# Autodesk Inventor assembly: complete
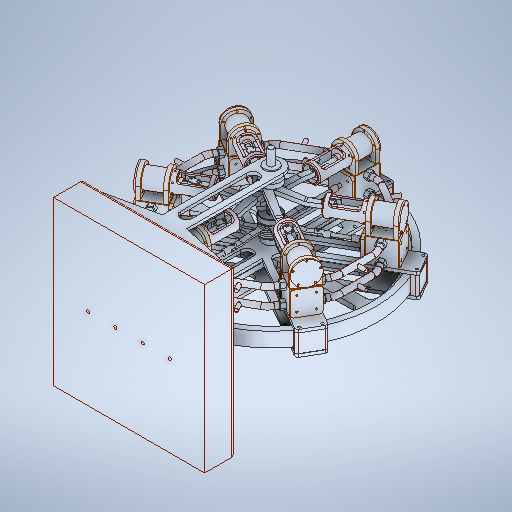
[picture p0: Inventor's stored thumbnail of the model, 512x512]
Saved by Autodesk Inventor 2025.1 (Build 291241000, 241)
## iProperties
Created: 2024-09-18
Part Number: complete
Document SubType Name: Assembly
Designer: ffogue
Author: ffogue
## Documents named in this file (23)
- C:\Users\ffogue\Documents\Inventor\Cylinder Radial Steam Engine\complete.iam
- C:\Users\ffogue\Documents\Inventor\Cylinder Radial Steam Engine\03.ipt
- C:\Users\ffogue\Documents\Inventor\Cylinder Radial Steam Engine\02A.ipt
- C:\Users\ffogue\Documents\Inventor\Cylinder Radial Steam Engine\05.ipt
- C:\Users\ffogue\Documents\Inventor\Cylinder Radial Steam Engine\04.ipt
- C:\Users\ffogue\Documents\Inventor\Cylinder Radial Steam Engine\08.ipt
- C:\Users\ffogue\Documents\Inventor\Cylinder Radial Steam Engine\09.ipt
- C:\Users\ffogue\Documents\Inventor\Cylinder Radial Steam Engine\Block.ipt
- C:\Users\ffogue\Documents\Inventor\Cylinder Radial Steam Engine\02.ipt
- C:\Users\ffogue\Documents\Inventor\Cylinder Radial Steam Engine\03A.ipt
- C:\Users\ffogue\Documents\Inventor\Cylinder Radial Steam Engine\block.iam
- C:\Users\ffogue\Documents\Inventor\Cylinder Radial Steam Engine\51.ipt
- C:\Users\ffogue\Documents\Inventor\Cylinder Radial Steam Engine\axis.iam
- C:\Users\ffogue\Documents\Inventor\Cylinder Radial Steam Engine\axis assembly.iam
- C:\Users\ffogue\Documents\Inventor\Cylinder Radial Steam Engine\15_3.iam
- C:\Users\ffogue\Documents\Inventor\Cylinder Radial Steam Engine\15_2.iam
- C:\Users\ffogue\Documents\Inventor\Cylinder Radial Steam Engine\15_1.iam
- C:\Users\ffogue\Documents\Inventor\Cylinder Radial Steam Engine\11.ipt
- C:\Users\ffogue\Documents\Inventor\Cylinder Radial Steam Engine\12.ipt
- C:\Users\ffogue\Documents\Inventor\Cylinder Radial Steam Engine\47.ipt
- C:\Users\ffogue\Documents\Inventor\Cylinder Radial Steam Engine\47B.ipt
- C:\Users\ffogue\Documents\Inventor\Cylinder Radial Steam Engine\47A.ipt
- C:\Users\ffogue\Documents\Inventor\Cylinder Radial Steam Engine\Welle.iam
## Components (68 placed, 22 different names)
1. 03:1 — Mate:1, Mate:3, Insert:2, Mate:14, Mate:18, Insert:12, Insert:13, Insert:14, Mate:27, Insert:21, Mate:109, Insert:38
2. 03:2 — Mate:1, Flush:1, Flush:2, Mate:2, Insert:1, Mate:4, Mate:15, Mate:16, Mate:17, Mate:22, Mate:23, Insert:11, Mate:24, Mate:25, Mate:26, Insert:15, Insert:20, Mate:110, Insert:39
3. 02A:1 — Flush:1, Flush:2, Mate:2, Insert:1, Mate:3, Insert:2
4. 05:1 — Mate:4, Mate:5, Mate:6, Insert:5, Insert:6, Mate:7, Mate:8, Angle:1, Rotation:1, Rotation:2
5. 08:1 — Mate:6, Insert:5, Mate:8, Mate:9, Mate:10, Mate:11, Mate:12, Flush:3, Flush:4, Flush:5, Flush:6, Insert:22
6. 08:2 — Mate:5, Insert:6, Mate:7
7. 09:1 — Mate:9, Flush:6
8. 09:2 — Mate:10, Flush:4
9. 09:3 — Mate:12, Flush:3
10. 09:4 — Mate:11, Flush:5
11. Block:1 — Mate:13, Insert:7, Angle:2
12. 02:1 — Mate:13, Insert:7, Mate:14, Mate:15, Mate:16, Mate:17, Mate:18, Mate:19, Insert:8
13. 03A:1 — Mate:19, Insert:8, Insert:10, Mate:148, Insert:54
14. 04:3 — Insert:10
15. 02A:2 — Mate:24, Insert:12
16. 02A:3 — Mate:25, Insert:13
17. 02A:4 — Mate:27, Insert:15
18. 02A:5 — Mate:26, Insert:14
19. 04:5 — Insert:21
20. 04:6 — Insert:20, Insert:22
21. axis:1 [sub-assembly] — Mate:61, Mate:130, Insert:45
22. axis assembly:1 [sub-assembly] — Mate:66, Mate:104, Insert:35
23. axis assembly:2 [sub-assembly] — Mate:75, Mate:99, Insert:33
24. axis assembly:3 [sub-assembly] — Mate:77, Mate:108, Insert:37
25. axis assembly:4 [sub-assembly] — Mate:80, Mate:97, Insert:32
26. axis assembly:5 [sub-assembly] — Mate:89, Mate:95, Insert:31
27. 15_3:2 [sub-assembly] — Mate:95, Insert:31, Mate:96, Mate:105, Mate:107
28. 15_3:3 [sub-assembly] — Mate:96, Mate:97, Insert:32, Mate:98, Mate:103, Mate:113, Insert:42
29. 15_2:1 [sub-assembly] — Mate:98, Mate:99, Insert:33
30. axis assembly:6 [sub-assembly] — Mate:101, Mate:106, Insert:36
31. 15_1:2 [sub-assembly] — Mate:103, Mate:104, Insert:35
32. 15_1:3 [sub-assembly] — Mate:105, Mate:106, Insert:36
33. 15_2:2 [sub-assembly] — Mate:107, Mate:108, Insert:37
34. 08:3 — Mate:109, Insert:38
35. 08:4 — Mate:110, Insert:39, Mate:114, Mate:150
36. 11:1 — Mate:111, Mate:112, Insert:40, Insert:41, Mate:113, Mate:114
37. 12:1 — Mate:112, Insert:41, Insert:42, Mate:116, Mate:149
38. 12:2 — Mate:111, Insert:40, Mate:116, Rotation:2
39. axis:2 [sub-assembly] — Mate:117, Mate:133, Insert:51
40. axis:3 [sub-assembly] — Mate:118, Mate:143, Insert:52
41. axis:4 [sub-assembly] — Mate:119, Mate:129, Insert:44
42. axis:5 [sub-assembly] — Mate:120, Mate:141, Insert:50
43. axis:6 [sub-assembly] — Mate:121, Mate:145, Insert:53
44. 47:1 — Mate:123, Mate:129, Insert:44
45. 47:2 — Mate:123, Mate:130, Insert:45, Mate:140
46. 47B:1 — Mate:133, Insert:51, Mate:142
47. 47B:2 — Mate:140, Mate:141, Insert:50, Mate:144
48. 47A:1 — Mate:142, Mate:143, Insert:52, Mate:146, Mate:147
49. 47A:2 — Mate:144, Mate:145, Insert:53, Mate:146
50. Welle:1 [sub-assembly] — Mate:147, Mate:148, Mate:149, Insert:54, Mate:150, Rotation:1
51. block:1 [sub-assembly] — Mate:22, Mate:23, Insert:11, Mate:101, Mate:119
52. block:2 [sub-assembly] — Mate:89, Mate:120
53. block:3 [sub-assembly] — Mate:77, Mate:121
54. block:4 [sub-assembly] — Mate:61, Mate:66
55. block:5 [sub-assembly] — Mate:45, Mate:47, Mate:80, Mate:117
56. block:6 [sub-assembly] — Mate:44, Mate:46, Mate:75, Mate:118
57. 51:2 — Mate:46, Mate:47
58. 51:1 — Mate:44, Mate:45
59. 51:3
60. 51:4
61. 51:5
62. 51:6
63. 51:7
64. 51:8
65. 51:9
66. 51:10
67. 51:11
68. 51:12
## Component patterns: (6 elements, first: block:1), (6 elements, first: 51:2 + 51:1)
## Relationships (117: Mate 74, Insert 33, Flush 6, Angle 2, RelateRotation 2)
- Mate:1: 03:1 ↔ 03:2
- Flush:1: 03:2 ↔ 02A:1
- Flush:2: 03:2 ↔ 02A:1
- Mate:2: 03:2 ↔ 02A:1
- Insert:1: 03:2 ↔ 02A:1
- Mate:3: 03:1 ↔ 02A:1
- Insert:2: 03:1 ↔ 02A:1
- Mate:4: 03:2 ↔ 05:1
- Mate:5: 05:1 ↔ 08:2
- Mate:6: 05:1 ↔ 08:1
- Insert:5: 05:1 ↔ 08:1
- Insert:6: 05:1 ↔ 08:2
- Mate:7: 05:1 ↔ 08:2
- Mate:8: 05:1 ↔ 08:1
- Mate:9: 08:1 ↔ 09:1
- Mate:10: 08:1 ↔ 09:2
- Mate:11: 08:1 ↔ 09:4
- Mate:12: 08:1 ↔ 09:3
- Flush:3: 08:1 ↔ 09:3
- Flush:4: 08:1 ↔ 09:2
- Flush:5: 08:1 ↔ 09:4
- Flush:6: 08:1 ↔ 09:1
- Mate:13: Block:1 ↔ 02:1
- Insert:7: Block:1 ↔ 02:1
- Mate:14: 03:1 ↔ 02:1
- Mate:15: 03:2 ↔ 02:1
- Mate:16: 03:2 ↔ 02:1
- Mate:17: 03:2 ↔ 02:1
- Mate:18: 03:1 ↔ 02:1
- Mate:19: 02:1 ↔ 03A:1
- Insert:8: 02:1 ↔ 03A:1
- Insert:10: 03A:1 ↔ 04:3
- Mate:22: 03:2 ↔ block:1
- Mate:23: 03:2 ↔ block:1
- Insert:11: 03:2 ↔ block:1
- Mate:24: 03:2 ↔ 02A:2
- Insert:12: 03:1 ↔ 02A:2
- Mate:25: 03:2 ↔ 02A:3
- Insert:13: 03:1 ↔ 02A:3
- Mate:26: 03:2 ↔ 02A:5
- Insert:14: 03:1 ↔ 02A:5
- Mate:27: 03:1 ↔ 02A:4
- Insert:15: 03:2 ↔ 02A:4
- Insert:20: 03:2 ↔ 04:6
- Insert:21: 03:1 ↔ 04:5
- Mate:44: block:6 ↔ 51:1
- Mate:45: block:5 ↔ 51:1
- Mate:46: block:6 ↔ 51:2
- Mate:47: block:5 ↔ 51:2
- Insert:22: 08:1 ↔ 04:6
- Mate:61: axis:1 ↔ block:4
- Mate:66: axis assembly:1 ↔ block:4
- Mate:75: axis assembly:2 ↔ block:6
- Mate:77: axis assembly:3 ↔ block:3
- Mate:80: axis assembly:4 ↔ block:5
- Mate:89: axis assembly:5 ↔ block:2
- Mate:95: axis assembly:5 ↔ 15_3:2
- Insert:31: axis assembly:5 ↔ 15_3:2
- Mate:96: 15_3:2 ↔ 15_3:3
- Mate:97: axis assembly:4 ↔ 15_3:3
- Insert:32: axis assembly:4 ↔ 15_3:3
- Mate:98: 15_3:3 ↔ 15_2:1
- Mate:99: axis assembly:2 ↔ 15_2:1
- Insert:33: axis assembly:2 ↔ 15_2:1
- Mate:101: axis assembly:6 ↔ block:1
- Mate:103: 15_3:3 ↔ 15_1:2
- Mate:104: axis assembly:1 ↔ 15_1:2
- Insert:35: axis assembly:1 ↔ 15_1:2
- Mate:105: 15_3:2 ↔ 15_1:3
- Mate:106: axis assembly:6 ↔ 15_1:3
- Insert:36: axis assembly:6 ↔ 15_1:3
- Mate:107: 15_3:2 ↔ 15_2:2
- Mate:108: axis assembly:3 ↔ 15_2:2
- Insert:37: axis assembly:3 ↔ 15_2:2
- Mate:109: 03:1 ↔ 08:3
- Insert:38: 03:1 ↔ 08:3
- Mate:110: 03:2 ↔ 08:4
- Insert:39: 03:2 ↔ 08:4
- Mate:111: 11:1 ↔ 12:2
- Mate:112: 11:1 ↔ 12:1
- Insert:40: 11:1 ↔ 12:2
- Insert:41: 11:1 ↔ 12:1
- Mate:113: 15_3:3 ↔ 11:1
- Mate:114: 08:4 ↔ 11:1
- Insert:42: 15_3:3 ↔ 12:1
- Mate:116: 12:1 ↔ 12:2
- Mate:117: axis:2 ↔ block:5
- Mate:118: axis:3 ↔ block:6
- Mate:119: axis:4 ↔ block:1
- Mate:120: axis:5 ↔ block:2
- Mate:121: axis:6 ↔ block:3
- Mate:123: 47:1 ↔ 47:2
- Mate:129: axis:4 ↔ 47:1
- Insert:44: axis:4 ↔ 47:1
- Mate:130: axis:1 ↔ 47:2
- Insert:45: axis:1 ↔ 47:2
- Mate:133: axis:2 ↔ 47B:1
- Mate:140: 47:2 ↔ 47B:2
- Mate:141: axis:5 ↔ 47B:2
- Insert:50: axis:5 ↔ 47B:2
- Insert:51: axis:2 ↔ 47B:1
- Mate:142: 47B:1 ↔ 47A:1
- Mate:143: axis:3 ↔ 47A:1
- Insert:52: axis:3 ↔ 47A:1
- Mate:144: 47B:2 ↔ 47A:2
- Mate:145: axis:6 ↔ 47A:2
- Insert:53: axis:6 ↔ 47A:2
- Mate:146: 47A:1 ↔ 47A:2
- Mate:147: 47A:1 ↔ Welle:1
- Mate:148: 03A:1 ↔ Welle:1
- Mate:149: 12:1 ↔ Welle:1
- Insert:54 (10 mm): 03A:1 ↔ Welle:1
- Angle:1 (0 deg): 05:1
- Mate:150: 08:4 ↔ Welle:1
- Rotation:1 [RelateRotation] (1 ul): 05:1 ↔ Welle:1
- Rotation:2 [RelateRotation] (2 ul): 05:1 ↔ 12:2
- Angle:2 (0 deg): Block:1
